# Autodesk Inventor assembly: obudowa - dzwonek
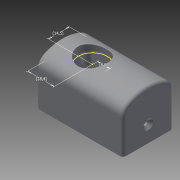
[picture p0: Inventor's stored thumbnail of the model, 180x180]
Saved by Autodesk Inventor 2014 (Build 180170000, 170)
## iProperties
Created: 2018-02-28
Part Number: obudowa - dzwonek
Document SubType Name: Assembly
Designer: HP820
Author: HP820
## Documents named in this file (3)
- C:\Users\HP820\Dysk Google\Projekt SYSTEM POWIADOMIEN DLA OSOB GLUCHONIEMYCH I NIEDOSLYSZACYCH BY JACEK MARTYNIAK I ŁUKASZ NOWARKIEWICZ\Projekty 3D obudowy\obudowa - dzwonek\obudowa - dzwonek.iam
- C:\Users\HP820\Dysk Google\Projekt SYSTEM POWIADOMIEN DLA OSOB GLUCHONIEMYCH I NIEDOSLYSZACYCH BY JACEK MARTYNIAK I ŁUKASZ NOWARKIEWICZ\Projekty 3D obudowy\obudowa - dzwonek\obudowa - dzwonek - front.ipt
- C:\Users\HP820\Dysk Google\Projekt SYSTEM POWIADOMIEN DLA OSOB GLUCHONIEMYCH I NIEDOSLYSZACYCH BY JACEK MARTYNIAK I ŁUKASZ NOWARKIEWICZ\Projekty 3D obudowy\obudowa - dzwonek\obudowa - dzwonek- tyl mocowanie do sciany.ipt
## Components (2 placed, 2 different names)
1. obudowa - dzwonek - front:1 — Flush:1
2. obudowa - dzwonek- tyl mocowanie do sciany:1 — Flush:1
## Relationships (1: Flush 1)
- Flush:1: obudowa - dzwonek - front:1 ↔ obudowa - dzwonek- tyl mocowanie do sciany:1
